# Autodesk Inventor assembly: AssemblyFullPrinter
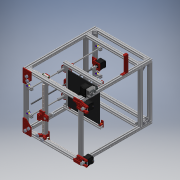
[picture p0: Inventor's stored thumbnail of the model, 180x180]
Saved by Autodesk Inventor 2018 (Build 220112000, 112)
## iProperties
Created: 2017-10-01
Part Number: AssemblyFullPrinter
Document SubType Name: Assembly
Designer: Jurjen
Author: Jurjen
## Documents named in this file (42)
- C:\Users\Jurjen\Documents\3D Printer\coreXY\AssemblyFullPrinter.iam
- C:\Users\Jurjen\Documents\3D Printer\coreXY\2020-350mm.ipt
- C:\Users\Jurjen\Documents\3D Printer\coreXY\2020-500mm.ipt
- C:\Users\Jurjen\Documents\3D Printer\coreXY\2020-corner-bracket.ipt
- C:\Users\Jurjen\Documents\3D Printer\coreXY\heated-bed.ipt
- C:\Users\Jurjen\Documents\3D Printer\coreXY\T8-lead-screw.ipt
- C:\Users\Jurjen\Documents\3D Printer\coreXY\motedis\GT2-Pulley-20-Teeth-5mm-Bore.ipt
- C:\Users\Jurjen\Documents\3D Printer\coreXY\motedis\Gt20.ipt
- C:\Users\Jurjen\Documents\3D Printer\coreXY\motedis\shaft-couple-flex.ipt
- C:\Users\Jurjen\Documents\3D Printer\coreXY\motedis\Motedis_SH8.ipt
- C:\Users\Jurjen\Documents\3D Printer\coreXY\rod-8mm.ipt
- C:\Users\Jurjen\Documents\3D Printer\coreXY\2020-260mm.ipt
- C:\Users\Jurjen\Documents\3D Printer\coreXY\2020-240mm.ipt
- C:\Users\Jurjen\Documents\3D Printer\coreXY\T8x2mm lead screw.ipt
- C:\Users\Jurjen\Documents\3D Printer\coreXY\OldhamCouplerBottom.ipt
- C:\Users\Jurjen\Documents\3D Printer\coreXY\OldhamCouplerMiddle.ipt
- C:\Users\Jurjen\Documents\3D Printer\coreXY\OldhamCouplerTop.ipt
- C:\Users\Jurjen\Documents\3D Printer\coreXY\M5-nut.ipt
- C:\Users\Jurjen\Documents\3D Printer\coreXY\nema17-mount-bottom-z-axis.ipt
- C:\Users\Jurjen\Documents\3D Printer\coreXY\bracket-GT2-left.ipt
- C:\Users\Jurjen\Documents\3D Printer\coreXY\M5x30mm.ipt
- C:\Users\Jurjen\Documents\3D Printer\coreXY\mount-heated-bed.ipt
- C:\Users\Jurjen\Documents\3D Printer\coreXY\bracket-GT2-right.ipt
- C:\Users\Jurjen\Documents\3D Printer\coreXY\spool-holder.ipt
- C:\Users\Jurjen\Documents\3D Printer\coreXY\17HM15-0904S\nema-17.ipt
- C:\Users\Jurjen\Documents\3D Printer\coreXY\nema17-mount-left.ipt
- C:\Users\Jurjen\Documents\3D Printer\coreXY\nema17-mount-right.ipt
- C:\Users\Jurjen\Documents\3D Printer\coreXY\LMF8LUU.ipt
- C:\Users\Jurjen\Documents\3D Printer\coreXY\holder-LMF8LUU-z-axis.ipt
- C:\Users\Jurjen\Documents\3D Printer\coreXY\MGN-12-rail.ipt
- C:\Users\Jurjen\Documents\3D Printer\coreXY\2020-320mm.ipt
- C:\Users\Jurjen\Documents\3D Printer\coreXY\x-carriage-2020.ipt
- C:\Users\Jurjen\Documents\3D Printer\coreXY\X-connectorLeft.ipt
- C:\Users\Jurjen\Documents\3D Printer\coreXY\X-connectorLeft_MIR.ipt
- C:\Users\Jurjen\Documents\3D Printer\coreXY\MGN-12-H-carriage.ipt
- C:\Users\Jurjen\Documents\3D Printer\coreXY\ED3V6.ipt
- C:\Users\Jurjen\Documents\3D Printer\coreXY\x-carriage.ipt
- C:\Users\Jurjen\Documents\3D Printer\coreXY\x-carriage-holder.ipt
- C:\Users\Jurjen\Documents\3D Printer\coreXY\holder-GT2-x-carriage-left.ipt
- C:\Users\Jurjen\Documents\3D Printer\coreXY\M5x35mm-crosshead.ipt
- C:\Users\Jurjen\Documents\3D Printer\coreXY\extruder\e3d titan.iam
- C:\Users\Jurjen\Documents\3D Printer\coreXY\mount-extruder.ipt
## Components (122 placed, 41 different names)
1. spool-holder:1 — Mate:287, Mate:288, Flush:54
2. 2020-500mm:1 — Mate:1, Flush:2, Flush:14, Flush:17, Mate:11, Mate:85, Flush:37, Mate:90, Mate:92, Mate:93, Mate:94, Mate:131, Mate:132, Mate:163, Mate:165, Mate:166, Mate:168, Mate:287, Mate:288, Flush:54, Mate:348, Mate:359, Mate:360, Mate:434, Flush:78, Mate:459, Mate:471, Mate:472, Mate:473
3. 2020-500mm:2 — Mate:2, Flush:1, Flush:13, Flush:14, Mate:12, Flush:23, Mate:75, Mate:77, Mate:79, Mate:80, Mate:133, Mate:135, Mate:151, Mate:152, Mate:154, Mate:156, Mate:346, Flush:63, Mate:362, Mate:439, Mate:455
4. 2020-500mm:3 — Mate:8, Flush:12, Flush:13, Flush:15, Mate:9, Flush:30, Mate:82, Mate:83, Mate:86, Flush:39, Mate:136, Mate:138, Mate:140, Mate:141, Mate:149, Mate:150, Mate:342, Flush:62, Flush:67, Mate:367, Flush:82, Mate:456
5. 2020-500mm:4 — Mate:7, Flush:15, Mate:10, Flush:27, Mate:142, Mate:144, Mate:145, Mate:147, Mate:157, Mate:158, Mate:160, Mate:162, Flush:64, Mate:354, Flush:65, Mate:447, Mate:450
6. 2020-320mm:3 — Mate:353, Mate:354, Mate:355, Mate:356, Flush:65, Flush:66, Mate:357, Mate:358, Mate:368, Mate:369, Mate:373, Mate:374, Mate:388, Flush:73, Mate:446, Mate:448, Mate:460, Mate:461
7. 2020-320mm:4 — Flush:67, Mate:362, Mate:363, Mate:364, Flush:68, Mate:366, Flush:69, Mate:371, Mate:372, Mate:385, Mate:386, Mate:387, Flush:72, Mate:453, Mate:454, Mate:457, Mate:458
8. 2020-350mm:1 — Mate:1, Mate:2, Flush:1, Flush:2, Mate:19, Mate:23, Mate:76, Mate:95, Mate:294, Mate:303, Mate:304, Mate:307, Mate:308, Flush:66, Flush:68
9. 2020-350mm:4 — Mate:7, Mate:8, Flush:12, Mate:16, Mate:26, Flush:27, Mate:60, Mate:61, Mate:64, Mate:65, Mate:66, Mate:67, Mate:239, Mate:277, Mate:279, Flush:53, Mate:337, Flush:70, Mate:449, Mate:452
10. 2020-corner-bracket:1 — Mate:16, Mate:356, Mate:452
11. 2020-corner-bracket:2 — Mate:23, Mate:363, Mate:364
12. 2020-corner-bracket:3 — Mate:19, Mate:357, Mate:358
13. 2020-corner-bracket:4 — Mate:26, Mate:385, Mate:386
14. 2020-corner-bracket:10 — Mate:75, Mate:76, Mate:77
15. 2020-corner-bracket:13 — Mate:93, Mate:94, Mate:95, Mate:359
16. 2020-corner-bracket:33 — Mate:449, Mate:450
17. 2020-corner-bracket:34 — Mate:446, Mate:447, Mate:448
18. 2020-corner-bracket:35 — Mate:453, Mate:454, Mate:455
19. 2020-corner-bracket:36 — Mate:456, Mate:457, Mate:458
20. 2020-corner-bracket:37 — Mate:459, Mate:460, Mate:461
21. 2020-320mm:1 — Mate:347, Flush:64, Mate:348, Mate:349, Mate:350, Mate:351, Mate:352
22. 2020-320mm:2 — Mate:338, Mate:339, Mate:341, Flush:61, Mate:342, Mate:343, Mate:344, Flush:62, Mate:345, Mate:346, Flush:63, Mate:445
23. 2020-350mm:5 — Flush:17, Mate:11, Mate:12, Mate:31, Mate:35, Flush:23, Mate:78, Mate:89, Mate:91, Mate:340, Flush:61
24. 2020-350mm:6 — Mate:9, Mate:10, Mate:27, Mate:28, Mate:29, Mate:30, Mate:34, Mate:38, Flush:30, Mate:62, Mate:63, Mate:68, Mate:69, Mate:70, Mate:71, Mate:72, Mate:139, Mate:146, Mate:230, Flush:59, Flush:60
25. 2020-corner-bracket:5 — Mate:27, Mate:38, Mate:351
26. 2020-corner-bracket:6 — Mate:28, Mate:34, Mate:343, Mate:345
27. 2020-corner-bracket:7 — Mate:30, Mate:35, Mate:338, Mate:339, Mate:340
28. 2020-corner-bracket:8 — Mate:29, Mate:31, Mate:349
29. 2020-corner-bracket:9 — Mate:78, Mate:79, Mate:80
30. 2020-corner-bracket:11 — Mate:82, Mate:83, Mate:344
31. 2020-corner-bracket:12 — Mate:89, Mate:90, Mate:91, Mate:92
32. 2020-corner-bracket:16 — Mate:139, Mate:140, Mate:141
33. 2020-corner-bracket:21 — Mate:145, Mate:146, Mate:147
34. 2020-corner-bracket:23 — Mate:151, Mate:152, Mate:341
35. 2020-corner-bracket:25 — Mate:157, Mate:158, Mate:347, Mate:352
36. 2020-corner-bracket:28 — Mate:166, Mate:168, Mate:350
37. 2020-350mm:10 — Mate:85, Flush:37, Mate:130, Mate:134, Mate:169, Mate:171, Mate:178, Mate:181, Flush:79
38. 2020-350mm:11 — Mate:86, Flush:39, Mate:137, Mate:143, Mate:174, Mate:176, Mate:179, Flush:80, Flush:81
39. 2020-320mm:5 — Mate:434, Mate:435, Flush:78, Mate:436, Flush:79, Flush:80, Mate:437, Mate:438, Mate:444
40. 2020-320mm:6 — Flush:81, Mate:439, Mate:440, Mate:441, Flush:82, Mate:442, Mate:443, Mate:445
41. 2020-corner-bracket:17 — Mate:133, Mate:134, Mate:135
42. 2020-corner-bracket:18 — Mate:130, Mate:131, Mate:132
43. 2020-corner-bracket:19 — Mate:136, Mate:137, Mate:138
44. 2020-corner-bracket:20 — Mate:142, Mate:143, Mate:144
45. 2020-corner-bracket:22 — Mate:149, Mate:150, Mate:442
46. 2020-corner-bracket:24 — Mate:154, Mate:156, Mate:440
47. 2020-corner-bracket:26 — Mate:160, Mate:162, Mate:437
48. 2020-corner-bracket:27 — Mate:163, Mate:165, Mate:436
49. 2020-corner-bracket:29 — Mate:169, Mate:178, Mate:441
50. 2020-corner-bracket:30 — Mate:171, Mate:181, Mate:435
51. 2020-corner-bracket:31 — Mate:174, Mate:438, Mate:444
52. 2020-corner-bracket:32 — Mate:176, Mate:179, Mate:443
53. 2020-corner-bracket:14 — Mate:122, Mate:123, Mate:124
54. 2020-corner-bracket:15 — Mate:119, Mate:120, Mate:121, Flush:49
55. shaft-couple-flex:1 — Mate:59, Mate:114, Mate:293
56. LMF8LUU:1 — Mate:313, Mate:317, Mate:318, Mate:320
57. LMF8LUU:2 — Mate:314, Mate:324, Mate:326, Mate:327
58. holder-LMF8LUU-z-axis:1 — Mate:316, Mate:317, Mate:318, Mate:319, Mate:320, Mate:321, Mate:322
59. holder-LMF8LUU-z-axis:2 — Mate:324, Mate:326, Mate:327, Mate:328, Mate:329, Mate:332
60. T8-lead-screw:1 — Mate:59, Mate:114, Mate:115, Mate:116, Mate:117, Mate:118, Mate:315
61. nema-17:1 — Mate:290, Mate:291, Mate:292, Mate:293, Mate:315
62. nema17-mount-bottom-z-axis:1 — Mate:230, Mate:290, Mate:291, Mate:292, Flush:59, Flush:60, Mate:330, Mate:331
63. rod-8mm:1 — Mate:73, Flush:34, Mate:314
64. rod-8mm:2 — Mate:74, Flush:35, Mate:313, Mate:316
65. heated-bed:1 — Mate:267, Mate:269, Mate:272, Mate:275, Mate:276
66. 2020-260mm:1 — Mate:109, Flush:45, Flush:46, Mate:123, Mate:265, Mate:266, Flush:52, Mate:270, Mate:271
67. 2020-260mm:2 — Mate:107, Flush:45, Flush:47, Mate:119, Flush:49, Mate:263, Mate:264, Flush:51, Mate:273, Mate:274
68. 2020-240mm:1 — Mate:103, Mate:104, Mate:105, Mate:107, Mate:109, Flush:46, Flush:47, Mate:110, Mate:120, Mate:121, Mate:122, Mate:124, Mate:319, Mate:321, Mate:322, Mate:328, Mate:329, Mate:332
69. mount-heated-bed:1 — Mate:263, Mate:264, Flush:51, Mate:267, Mate:276
70. mount-heated-bed:2 — Mate:265, Mate:266, Flush:52, Mate:269
71. mount-heated-bed:3 — Mate:270, Mate:271, Mate:272
72. mount-heated-bed:4 — Mate:273, Mate:274, Mate:275
73. Gt20:7 — Mate:424, Mate:433, Flush:76
74. Gt20:8 — Mate:423, Mate:427, Flush:77
75. MGN-12-rail:2 — Mate:373, Mate:374, Mate:388, Mate:394, Mate:395, Flush:73
76. MGN-12-rail:3 — Mate:371, Mate:372, Mate:387, Mate:392, Mate:393, Flush:72
77. MGN-12-H-carriage:1 — Mate:392, Mate:393, Mate:399, Mate:415
78. MGN-12-H-carriage:3 — Mate:394, Mate:395, Mate:396, Mate:397, Mate:398
79. GT2-Pulley-20-Teeth-5mm-Bore:2 — Mate:312, Flush:75
80. GT2-Pulley-20-Teeth-5mm-Bore:1 — Mate:297, Flush:56
81. bracket-GT2-right:1 — Mate:277, Mate:279, Mate:280, Mate:281, Mate:283, Mate:284, Mate:285, Mate:286, Flush:53, Mate:353, Mate:355
82. Gt20:5 — Mate:240, Mate:241, Flush:56, Mate:419, Flush:77
83. Gt20:6 — Mate:242, Mate:243, Mate:262, Flush:76
84. M5-nut:6 — Mate:260, Mate:283
85. bracket-GT2-left:1 — Mate:237, Mate:238, Mate:239, Mate:245, Mate:247, Mate:262, Mate:366, Mate:367, Flush:70, Mate:419
86. M5-nut:3 — Mate:244, Mate:245
87. M5-nut:5 — Mate:246, Mate:247
88. M5x30mm:1 — Mate:237, Mate:240, Mate:241, Mate:244
89. M5x30mm:2 — Mate:238, Mate:242, Mate:243, Mate:246
90. M5x30mm:3 — Mate:254, Mate:256, Mate:260, Mate:281
91. M5x30mm:4 — Mate:255, Mate:257, Mate:258, Mate:280
92. Gt20:2 — Mate:254, Mate:256, Mate:286, Flush:75
93. Gt20:4 — Mate:255, Mate:257, Mate:285
94. M5-nut:2 — Mate:258, Mate:284
95. nema-17:2 — Mate:297, Mate:298, Mate:299, Mate:300, Flush:57
96. nema-17:3 — Mate:309, Mate:310, Flush:58, Mate:311, Mate:312
97. nema17-mount-left:1 — Mate:294, Mate:298, Mate:299, Mate:300, Flush:57, Mate:303, Mate:304, Flush:69
98. nema17-mount-right:1 — Mate:307, Mate:308, Mate:309, Mate:310, Flush:58, Mate:311, Mate:360, Mate:368, Mate:369
99. e3d titan:1 [sub-assembly] — Mate:465, Mate:466, Mate:470
100. mount-extruder:1 — Mate:465, Mate:466, Mate:467, Mate:468, Mate:469, Mate:470, Mate:471, Mate:472, Mate:473
101. nema-17:4 — Mate:467, Mate:468, Mate:469
102. Motedis_SH8:1 — Mate:63, Mate:71, Mate:72, Flush:33, Mate:331
103. Motedis_SH8:2 — Mate:62, Mate:68, Mate:69, Mate:70, Flush:32, Mate:330
104. Motedis_SH8:3 — Mate:61, Mate:64, Mate:65, Flush:33, Mate:74, Flush:35
105. Motedis_SH8:4 — Mate:60, Mate:66, Mate:67, Flush:32, Mate:73, Flush:34
106. T8x2mm lead screw:1 — Mate:100, Mate:118
107. OldhamCouplerBottom:1 — Mate:99, Flush:43, Mate:100, Mate:117
108. OldhamCouplerMiddle:1 — Mate:99, Flush:43, Flush:44, Mate:102, Mate:115
109. OldhamCouplerTop:1 — Flush:44, Mate:102, Mate:103, Mate:104, Mate:105, Mate:110, Mate:116, Mate:337
110. MGN-12-rail:1 — Mate:381, Mate:389, Mate:390, Mate:391, Flush:71
111. x-carriage-2020:1 — Mate:377, Mate:381, Mate:384, Mate:389, Flush:71, Mate:409, Mate:410, Mate:411, Mate:421, Mate:422, Mate:432
112. X-connectorLeft:1 — Mate:377, Mate:396, Mate:397, Mate:398, Mate:410, Mate:411
113. X-connectorLeft_MIR:1 — Mate:384, Mate:399, Mate:409, Mate:415
114. MGN-12-H-carriage:2 — Mate:390, Mate:391, Mate:402, Mate:403, Mate:404
115. x-carriage-holder:1 — Mate:406, Mate:407, Mate:408
116. x-carriage:1 — Mate:402, Mate:403, Mate:404, Mate:405, Mate:406, Mate:407, Mate:408, Flush:74
117. holder-GT2-x-carriage-left:1 — Mate:421, Mate:422, Mate:425, Mate:426, Mate:429, Mate:431, Mate:432
118. M5-nut:7 — Mate:428, Mate:429
119. M5x35mm-crosshead:1 — Mate:423, Mate:426, Mate:427, Mate:428
120. M5-nut:8 — Mate:430, Mate:431
121. M5x35mm-crosshead:2 — Mate:424, Mate:425, Mate:430, Mate:433
122. ED3V6:1 — Mate:405, Flush:74
## Relationships (356: Mate 303, Flush 53)
- Mate:1: 2020-500mm:1 ↔ 2020-350mm:1
- Mate:2: 2020-500mm:2 ↔ 2020-350mm:1
- Flush:1: 2020-500mm:2 ↔ 2020-350mm:1
- Flush:2: 2020-500mm:1 ↔ 2020-350mm:1
- Mate:7: 2020-500mm:4 ↔ 2020-350mm:4
- Mate:8: 2020-500mm:3 ↔ 2020-350mm:4
- Flush:12: 2020-500mm:3 ↔ 2020-350mm:4
- Flush:13: 2020-500mm:2 ↔ 2020-500mm:3
- Flush:14: 2020-500mm:1 ↔ 2020-500mm:2
- Flush:15: 2020-500mm:3 ↔ 2020-500mm:4
- Mate:9: 2020-500mm:3 ↔ 2020-350mm:6
- Mate:10: 2020-500mm:4 ↔ 2020-350mm:6
- Flush:17: 2020-500mm:1 ↔ 2020-350mm:5
- Mate:11: 2020-500mm:1 ↔ 2020-350mm:5
- Mate:12: 2020-500mm:2 ↔ 2020-350mm:5
- Mate:16: 2020-350mm:4 ↔ 2020-corner-bracket:1
- Mate:19: 2020-350mm:1 ↔ 2020-corner-bracket:3
- Mate:23: 2020-350mm:1 ↔ 2020-corner-bracket:2
- Mate:26: 2020-350mm:4 ↔ 2020-corner-bracket:4
- Mate:27: 2020-350mm:6 ↔ 2020-corner-bracket:5
- Mate:28: 2020-350mm:6 ↔ 2020-corner-bracket:6
- Mate:29: 2020-350mm:6 ↔ 2020-corner-bracket:8
- Mate:30: 2020-350mm:6 ↔ 2020-corner-bracket:7
- Mate:31: 2020-350mm:5 ↔ 2020-corner-bracket:8
- Mate:34: 2020-350mm:6 ↔ 2020-corner-bracket:6
- Mate:35: 2020-350mm:5 ↔ 2020-corner-bracket:7
- Mate:38: 2020-350mm:6 ↔ 2020-corner-bracket:5
- Flush:23: 2020-500mm:2 ↔ 2020-350mm:5
- Flush:27: 2020-500mm:4 ↔ 2020-350mm:4
- Flush:30: 2020-500mm:3 ↔ 2020-350mm:6
- Mate:59 (-8 mm): shaft-couple-flex:1 ↔ T8-lead-screw:1
- Mate:60: 2020-350mm:4 ↔ Motedis_SH8:4
- Mate:61: 2020-350mm:4 ↔ Motedis_SH8:3
- Mate:62: 2020-350mm:6 ↔ Motedis_SH8:2
- Mate:63: 2020-350mm:6 ↔ Motedis_SH8:1
- Mate:64: 2020-350mm:4 ↔ Motedis_SH8:3
- Mate:65: 2020-350mm:4 ↔ Motedis_SH8:3
- Mate:66: 2020-350mm:4 ↔ Motedis_SH8:4
- Mate:67: 2020-350mm:4 ↔ Motedis_SH8:4
- Mate:68: 2020-350mm:6 ↔ Motedis_SH8:2
- Mate:69: 2020-350mm:6 ↔ Motedis_SH8:2
- Mate:70: 2020-350mm:6 ↔ Motedis_SH8:2
- Flush:32: Motedis_SH8:2 ↔ Motedis_SH8:4
- Mate:71: 2020-350mm:6 ↔ Motedis_SH8:1
- Mate:72: 2020-350mm:6 ↔ Motedis_SH8:1
- Flush:33: Motedis_SH8:1 ↔ Motedis_SH8:3
- Mate:73: rod-8mm:1 ↔ Motedis_SH8:4
- Mate:74: rod-8mm:2 ↔ Motedis_SH8:3
- Flush:34 (-5 mm): rod-8mm:1 ↔ Motedis_SH8:4
- Flush:35 (-5 mm): rod-8mm:2 ↔ Motedis_SH8:3
- Mate:75: 2020-500mm:2 ↔ 2020-corner-bracket:10
- Mate:76: 2020-350mm:1 ↔ 2020-corner-bracket:10
- Mate:77: 2020-500mm:2 ↔ 2020-corner-bracket:10
- Mate:78: 2020-350mm:5 ↔ 2020-corner-bracket:9
- Mate:79: 2020-500mm:2 ↔ 2020-corner-bracket:9
- Mate:80: 2020-500mm:2 ↔ 2020-corner-bracket:9
- Mate:82: 2020-500mm:3 ↔ 2020-corner-bracket:11
- Mate:83: 2020-500mm:3 ↔ 2020-corner-bracket:11
- Mate:85: 2020-500mm:1 ↔ 2020-350mm:10
- Flush:37: 2020-500mm:1 ↔ 2020-350mm:10
- Mate:86: 2020-500mm:3 ↔ 2020-350mm:11
- Flush:39: 2020-500mm:3 ↔ 2020-350mm:11
- Mate:89: 2020-350mm:5 ↔ 2020-corner-bracket:12
- Mate:90: 2020-500mm:1 ↔ 2020-corner-bracket:12
- Mate:91: 2020-350mm:5 ↔ 2020-corner-bracket:12
- Mate:92: 2020-500mm:1 ↔ 2020-corner-bracket:12
- Mate:93: 2020-500mm:1 ↔ 2020-corner-bracket:13
- Mate:94: 2020-500mm:1 ↔ 2020-corner-bracket:13
- Mate:95: 2020-350mm:1 ↔ 2020-corner-bracket:13
- Mate:99: OldhamCouplerBottom:1 ↔ OldhamCouplerMiddle:1
- Flush:43: OldhamCouplerBottom:1 ↔ OldhamCouplerMiddle:1
- Mate:100: T8x2mm lead screw:1 ↔ OldhamCouplerBottom:1
- Flush:44: OldhamCouplerMiddle:1 ↔ OldhamCouplerTop:1
- Mate:102: OldhamCouplerMiddle:1 ↔ OldhamCouplerTop:1
- Mate:103: 2020-240mm:1 ↔ OldhamCouplerTop:1
- Mate:104: 2020-240mm:1 ↔ OldhamCouplerTop:1
- Mate:105: 2020-240mm:1 ↔ OldhamCouplerTop:1
- Mate:107: 2020-260mm:2 ↔ 2020-240mm:1
- Mate:109: 2020-260mm:1 ↔ 2020-240mm:1
- Flush:45: 2020-260mm:1 ↔ 2020-260mm:2
- Flush:46: 2020-260mm:1 ↔ 2020-240mm:1
- Flush:47: 2020-260mm:2 ↔ 2020-240mm:1
- Mate:110: 2020-240mm:1 ↔ OldhamCouplerTop:1
- Mate:114: shaft-couple-flex:1 ↔ T8-lead-screw:1
- Mate:115: T8-lead-screw:1 ↔ OldhamCouplerMiddle:1
- Mate:116: T8-lead-screw:1 ↔ OldhamCouplerTop:1
- Mate:117: T8-lead-screw:1 ↔ OldhamCouplerBottom:1
- Mate:118: T8-lead-screw:1 ↔ T8x2mm lead screw:1
- Mate:119: 2020-corner-bracket:15 ↔ 2020-260mm:2
- Mate:120: 2020-corner-bracket:15 ↔ 2020-240mm:1
- Mate:121: 2020-corner-bracket:15 ↔ 2020-240mm:1
- Flush:49: 2020-corner-bracket:15 ↔ 2020-260mm:2
- Mate:122: 2020-corner-bracket:14 ↔ 2020-240mm:1
- Mate:123: 2020-corner-bracket:14 ↔ 2020-260mm:1
- Mate:124: 2020-corner-bracket:14 ↔ 2020-240mm:1
- Mate:130: 2020-350mm:10 ↔ 2020-corner-bracket:18
- Mate:131: 2020-500mm:1 ↔ 2020-corner-bracket:18
- Mate:132: 2020-500mm:1 ↔ 2020-corner-bracket:18
- Mate:133: 2020-500mm:2 ↔ 2020-corner-bracket:17
- Mate:134: 2020-350mm:10 ↔ 2020-corner-bracket:17
- Mate:135: 2020-500mm:2 ↔ 2020-corner-bracket:17
- Mate:136: 2020-500mm:3 ↔ 2020-corner-bracket:19
- Mate:137: 2020-350mm:11 ↔ 2020-corner-bracket:19
- Mate:138: 2020-500mm:3 ↔ 2020-corner-bracket:19
- Mate:139: 2020-350mm:6 ↔ 2020-corner-bracket:16
- Mate:140: 2020-500mm:3 ↔ 2020-corner-bracket:16
- Mate:141: 2020-500mm:3 ↔ 2020-corner-bracket:16
- Mate:142: 2020-500mm:4 ↔ 2020-corner-bracket:20
- Mate:143: 2020-350mm:11 ↔ 2020-corner-bracket:20
- Mate:144: 2020-500mm:4 ↔ 2020-corner-bracket:20
- Mate:145: 2020-500mm:4 ↔ 2020-corner-bracket:21
- Mate:146: 2020-350mm:6 ↔ 2020-corner-bracket:21
- Mate:147: 2020-500mm:4 ↔ 2020-corner-bracket:21
- Mate:149: 2020-500mm:3 ↔ 2020-corner-bracket:22
- Mate:150: 2020-500mm:3 ↔ 2020-corner-bracket:22
- Mate:151: 2020-500mm:2 ↔ 2020-corner-bracket:23
- Mate:152: 2020-500mm:2 ↔ 2020-corner-bracket:23
- Mate:154: 2020-500mm:2 ↔ 2020-corner-bracket:24
- Mate:156: 2020-500mm:2 ↔ 2020-corner-bracket:24
- Mate:157: 2020-500mm:4 ↔ 2020-corner-bracket:25
- Mate:158: 2020-500mm:4 ↔ 2020-corner-bracket:25
- Mate:160: 2020-500mm:4 ↔ 2020-corner-bracket:26
- Mate:162: 2020-500mm:4 ↔ 2020-corner-bracket:26
- Mate:163: 2020-500mm:1 ↔ 2020-corner-bracket:27
- Mate:165: 2020-500mm:1 ↔ 2020-corner-bracket:27
- Mate:166: 2020-500mm:1 ↔ 2020-corner-bracket:28
- Mate:168: 2020-500mm:1 ↔ 2020-corner-bracket:28
- Mate:169: 2020-350mm:10 ↔ 2020-corner-bracket:29
- Mate:171: 2020-350mm:10 ↔ 2020-corner-bracket:30
- Mate:174: 2020-350mm:11 ↔ 2020-corner-bracket:31
- Mate:176: 2020-350mm:11 ↔ 2020-corner-bracket:32
- Mate:178: 2020-350mm:10 ↔ 2020-corner-bracket:29
- Mate:179: 2020-350mm:11 ↔ 2020-corner-bracket:32
- Mate:181: 2020-350mm:10 ↔ 2020-corner-bracket:30
- Mate:230: 2020-350mm:6 ↔ nema17-mount-bottom-z-axis:1
- Mate:237: bracket-GT2-left:1 ↔ M5x30mm:1
- Mate:238: bracket-GT2-left:1 ↔ M5x30mm:2
- Mate:239: 2020-350mm:4 ↔ bracket-GT2-left:1
- Mate:240: Gt20:5 ↔ M5x30mm:1
- Mate:241: Gt20:5 ↔ M5x30mm:1
- Mate:242: Gt20:6 ↔ M5x30mm:2
- Mate:243: Gt20:6 ↔ M5x30mm:2
- Mate:244: M5-nut:3 ↔ M5x30mm:1
- Mate:245: bracket-GT2-left:1 ↔ M5-nut:3
- Mate:246: M5-nut:5 ↔ M5x30mm:2
- Mate:247: bracket-GT2-left:1 ↔ M5-nut:5
- Mate:254: M5x30mm:3 ↔ Gt20:2
- Mate:255: M5x30mm:4 ↔ Gt20:4
- Mate:256: M5x30mm:3 ↔ Gt20:2
- Mate:257: M5x30mm:4 ↔ Gt20:4
- Mate:258: M5x30mm:4 ↔ M5-nut:2
- Mate:260: M5-nut:6 ↔ M5x30mm:3
- Mate:262: Gt20:6 ↔ bracket-GT2-left:1
- Mate:263: 2020-260mm:2 ↔ mount-heated-bed:1
- Mate:264: 2020-260mm:2 ↔ mount-heated-bed:1
- Flush:51: 2020-260mm:2 ↔ mount-heated-bed:1
- Mate:265: 2020-260mm:1 ↔ mount-heated-bed:2
- Mate:266: 2020-260mm:1 ↔ mount-heated-bed:2
- Flush:52: 2020-260mm:1 ↔ mount-heated-bed:2
- Mate:267: heated-bed:1 ↔ mount-heated-bed:1
- Mate:269: heated-bed:1 ↔ mount-heated-bed:2
- Mate:270: 2020-260mm:1 ↔ mount-heated-bed:3
- Mate:271: 2020-260mm:1 ↔ mount-heated-bed:3
- Mate:272: heated-bed:1 ↔ mount-heated-bed:3
- Mate:273: 2020-260mm:2 ↔ mount-heated-bed:4
- Mate:274: 2020-260mm:2 ↔ mount-heated-bed:4
- Mate:275: heated-bed:1 ↔ mount-heated-bed:4
- Mate:276 (20 mm): heated-bed:1 ↔ mount-heated-bed:1
- Mate:277: 2020-350mm:4 ↔ bracket-GT2-right:1
- Mate:279: 2020-350mm:4 ↔ bracket-GT2-right:1
- Mate:280: bracket-GT2-right:1 ↔ M5x30mm:4
- Mate:281: bracket-GT2-right:1 ↔ M5x30mm:3
- Mate:283: bracket-GT2-right:1 ↔ M5-nut:6
- Mate:284: bracket-GT2-right:1 ↔ M5-nut:2
- Mate:285: bracket-GT2-right:1 ↔ Gt20:4
- Mate:286: bracket-GT2-right:1 ↔ Gt20:2
- Flush:53: 2020-350mm:4 ↔ bracket-GT2-right:1
- Mate:287: spool-holder:1 ↔ 2020-500mm:1
- Mate:288: spool-holder:1 ↔ 2020-500mm:1
- Flush:54: spool-holder:1 ↔ 2020-500mm:1
- Mate:290: nema-17:1 ↔ nema17-mount-bottom-z-axis:1
- Mate:291: nema-17:1 ↔ nema17-mount-bottom-z-axis:1
- Mate:292: nema-17:1 ↔ nema17-mount-bottom-z-axis:1
- Mate:293 (-8 mm): shaft-couple-flex:1 ↔ nema-17:1
- Mate:294: 2020-350mm:1 ↔ nema17-mount-left:1
- Mate:297: GT2-Pulley-20-Teeth-5mm-Bore:1 ↔ nema-17:2
- Flush:56: GT2-Pulley-20-Teeth-5mm-Bore:1 ↔ Gt20:5
- Mate:298: nema-17:2 ↔ nema17-mount-left:1
- Mate:299: nema-17:2 ↔ nema17-mount-left:1
- Mate:300: nema-17:2 ↔ nema17-mount-left:1
- Flush:57: nema-17:2 ↔ nema17-mount-left:1
- Mate:303: 2020-350mm:1 ↔ nema17-mount-left:1
- Mate:304: 2020-350mm:1 ↔ nema17-mount-left:1
- Mate:307: 2020-350mm:1 ↔ nema17-mount-right:1
- Mate:308: 2020-350mm:1 ↔ nema17-mount-right:1
- Mate:309: nema-17:3 ↔ nema17-mount-right:1
- Mate:310: nema-17:3 ↔ nema17-mount-right:1
- Flush:58: nema-17:3 ↔ nema17-mount-right:1
- Mate:311: nema-17:3 ↔ nema17-mount-right:1
- Mate:312: GT2-Pulley-20-Teeth-5mm-Bore:2 ↔ nema-17:3
- Mate:313: LMF8LUU:1 ↔ rod-8mm:2
- Mate:314: LMF8LUU:2 ↔ rod-8mm:1
- Flush:59: 2020-350mm:6 ↔ nema17-mount-bottom-z-axis:1
- Flush:60: 2020-350mm:6 ↔ nema17-mount-bottom-z-axis:1
- Mate:315: T8-lead-screw:1 ↔ nema-17:1
- Mate:316: holder-LMF8LUU-z-axis:1 ↔ rod-8mm:2
- Mate:317: LMF8LUU:1 ↔ holder-LMF8LUU-z-axis:1
- Mate:318: LMF8LUU:1 ↔ holder-LMF8LUU-z-axis:1
- Mate:319: holder-LMF8LUU-z-axis:1 ↔ 2020-240mm:1
- Mate:320: LMF8LUU:1 ↔ holder-LMF8LUU-z-axis:1
- Mate:321: holder-LMF8LUU-z-axis:1 ↔ 2020-240mm:1
- Mate:322: holder-LMF8LUU-z-axis:1 ↔ 2020-240mm:1
- Mate:324: LMF8LUU:2 ↔ holder-LMF8LUU-z-axis:2
- Mate:326: LMF8LUU:2 ↔ holder-LMF8LUU-z-axis:2
- Mate:327: LMF8LUU:2 ↔ holder-LMF8LUU-z-axis:2
- Mate:328: holder-LMF8LUU-z-axis:2 ↔ 2020-240mm:1
- Mate:329: holder-LMF8LUU-z-axis:2 ↔ 2020-240mm:1
- Mate:330 (40 mm): nema17-mount-bottom-z-axis:1 ↔ Motedis_SH8:2
- Mate:331 (40 mm): nema17-mount-bottom-z-axis:1 ↔ Motedis_SH8:1
- Mate:332: holder-LMF8LUU-z-axis:2 ↔ 2020-240mm:1
- Mate:337: 2020-350mm:4 ↔ OldhamCouplerTop:1
- Mate:338: 2020-320mm:2 ↔ 2020-corner-bracket:7
- Mate:339: 2020-320mm:2 ↔ 2020-corner-bracket:7
- Mate:340: 2020-350mm:5 ↔ 2020-corner-bracket:7
- Mate:341: 2020-320mm:2 ↔ 2020-corner-bracket:23
- Flush:61: 2020-320mm:2 ↔ 2020-350mm:5
- Mate:342: 2020-500mm:3 ↔ 2020-320mm:2
- Mate:343: 2020-320mm:2 ↔ 2020-corner-bracket:6
- Mate:344: 2020-320mm:2 ↔ 2020-corner-bracket:11
- Flush:62: 2020-500mm:3 ↔ 2020-320mm:2
- Mate:345: 2020-320mm:2 ↔ 2020-corner-bracket:6
- Mate:346: 2020-500mm:2 ↔ 2020-320mm:2
- Flush:63: 2020-500mm:2 ↔ 2020-320mm:2
- Mate:347: 2020-320mm:1 ↔ 2020-corner-bracket:25
- Flush:64: 2020-500mm:4 ↔ 2020-320mm:1
- Mate:348: 2020-500mm:1 ↔ 2020-320mm:1
- Mate:349: 2020-320mm:1 ↔ 2020-corner-bracket:8
- Mate:350: 2020-320mm:1 ↔ 2020-corner-bracket:28
- Mate:351: 2020-320mm:1 ↔ 2020-corner-bracket:5
- Mate:352: 2020-320mm:1 ↔ 2020-corner-bracket:25
- Mate:353: 2020-320mm:3 ↔ bracket-GT2-right:1
- Mate:354: 2020-500mm:4 ↔ 2020-320mm:3
- Mate:355: 2020-320mm:3 ↔ bracket-GT2-right:1
- Mate:356: 2020-320mm:3 ↔ 2020-corner-bracket:1
- Flush:65: 2020-500mm:4 ↔ 2020-320mm:3
- Flush:66: 2020-320mm:3 ↔ 2020-350mm:1
- Mate:357: 2020-320mm:3 ↔ 2020-corner-bracket:3
- Mate:358: 2020-320mm:3 ↔ 2020-corner-bracket:3
- Mate:359: 2020-500mm:1 ↔ 2020-corner-bracket:13
- Mate:360: 2020-500mm:1 ↔ nema17-mount-right:1
- Flush:67: 2020-500mm:3 ↔ 2020-320mm:4
- Mate:362: 2020-500mm:2 ↔ 2020-320mm:4
- Mate:363: 2020-320mm:4 ↔ 2020-corner-bracket:2
- Mate:364: 2020-320mm:4 ↔ 2020-corner-bracket:2
- Flush:68: 2020-320mm:4 ↔ 2020-350mm:1
- Mate:366: 2020-320mm:4 ↔ bracket-GT2-left:1
- Mate:367: 2020-500mm:3 ↔ bracket-GT2-left:1
- Mate:368: 2020-320mm:3 ↔ nema17-mount-right:1
- Mate:369: 2020-320mm:3 ↔ nema17-mount-right:1
- Flush:69: 2020-320mm:4 ↔ nema17-mount-left:1
- Mate:371: 2020-320mm:4 ↔ MGN-12-rail:3
- Mate:372: 2020-320mm:4 ↔ MGN-12-rail:3
- Mate:373: 2020-320mm:3 ↔ MGN-12-rail:2
- Mate:374: 2020-320mm:3 ↔ MGN-12-rail:2
- Flush:70: 2020-350mm:4 ↔ bracket-GT2-left:1
- Mate:377: x-carriage-2020:1 ↔ X-connectorLeft:1
- Mate:381: MGN-12-rail:1 ↔ x-carriage-2020:1
- Mate:384: x-carriage-2020:1 ↔ X-connectorLeft_MIR:1
- Mate:385: 2020-320mm:4 ↔ 2020-corner-bracket:4
- Mate:386: 2020-320mm:4 ↔ 2020-corner-bracket:4
- Mate:387: 2020-320mm:4 ↔ MGN-12-rail:3
- Mate:388: 2020-320mm:3 ↔ MGN-12-rail:2
- Mate:389: MGN-12-rail:1 ↔ x-carriage-2020:1
- Mate:390: MGN-12-rail:1 ↔ MGN-12-H-carriage:2
- Mate:391: MGN-12-rail:1 ↔ MGN-12-H-carriage:2
- Mate:392: MGN-12-rail:3 ↔ MGN-12-H-carriage:1
- Mate:393: MGN-12-rail:3 ↔ MGN-12-H-carriage:1
- Mate:394: MGN-12-rail:2 ↔ MGN-12-H-carriage:3
- Mate:395: MGN-12-rail:2 ↔ MGN-12-H-carriage:3
- Mate:396: MGN-12-H-carriage:3 ↔ X-connectorLeft:1
- Mate:397: MGN-12-H-carriage:3 ↔ X-connectorLeft:1
- Mate:398: MGN-12-H-carriage:3 ↔ X-connectorLeft:1
- Mate:399: MGN-12-H-carriage:1 ↔ X-connectorLeft_MIR:1
- Flush:71: MGN-12-rail:1 ↔ x-carriage-2020:1
- Flush:72: 2020-320mm:4 ↔ MGN-12-rail:3
- Flush:73: 2020-320mm:3 ↔ MGN-12-rail:2
- Mate:402: MGN-12-H-carriage:2 ↔ x-carriage:1
- Mate:403: MGN-12-H-carriage:2 ↔ x-carriage:1
- Mate:404: MGN-12-H-carriage:2 ↔ x-carriage:1
- Mate:405: x-carriage:1 ↔ ED3V6:1
- Mate:406: x-carriage-holder:1 ↔ x-carriage:1
- Mate:407: x-carriage-holder:1 ↔ x-carriage:1
- Mate:408: x-carriage-holder:1 ↔ x-carriage:1
- Flush:74: x-carriage:1 ↔ ED3V6:1
- Flush:75: GT2-Pulley-20-Teeth-5mm-Bore:2 ↔ Gt20:2
- Mate:409: x-carriage-2020:1 ↔ X-connectorLeft_MIR:1
- Mate:410: x-carriage-2020:1 ↔ X-connectorLeft:1
- Mate:411 (-27 mm): x-carriage-2020:1 ↔ X-connectorLeft:1
- Mate:415: MGN-12-H-carriage:1 ↔ X-connectorLeft_MIR:1
- Mate:419: Gt20:5 ↔ bracket-GT2-left:1
- Mate:421: x-carriage-2020:1 ↔ holder-GT2-x-carriage-left:1
- Mate:422: x-carriage-2020:1 ↔ holder-GT2-x-carriage-left:1
- Mate:423: Gt20:8 ↔ M5x35mm-crosshead:1
- Mate:424: Gt20:7 ↔ M5x35mm-crosshead:2
- Mate:425: holder-GT2-x-carriage-left:1 ↔ M5x35mm-crosshead:2
- Mate:426: holder-GT2-x-carriage-left:1 ↔ M5x35mm-crosshead:1
- Mate:427: Gt20:8 ↔ M5x35mm-crosshead:1
- Mate:428: M5-nut:7 ↔ M5x35mm-crosshead:1
- Mate:429: holder-GT2-x-carriage-left:1 ↔ M5-nut:7
- Mate:430: M5-nut:8 ↔ M5x35mm-crosshead:2
- Mate:431: holder-GT2-x-carriage-left:1 ↔ M5-nut:8
- Mate:432: x-carriage-2020:1 ↔ holder-GT2-x-carriage-left:1
- Mate:433: Gt20:7 ↔ M5x35mm-crosshead:2
- Flush:76: Gt20:7 ↔ Gt20:6
- Flush:77: Gt20:8 ↔ Gt20:5
- Mate:434: 2020-500mm:1 ↔ 2020-320mm:5
- Mate:435: 2020-320mm:5 ↔ 2020-corner-bracket:30
- Flush:78: 2020-500mm:1 ↔ 2020-320mm:5
- Mate:436: 2020-320mm:5 ↔ 2020-corner-bracket:27
- Flush:79: 2020-350mm:10 ↔ 2020-320mm:5
- Flush:80: 2020-350mm:11 ↔ 2020-320mm:5
- Flush:81: 2020-350mm:11 ↔ 2020-320mm:6
- Mate:437: 2020-320mm:5 ↔ 2020-corner-bracket:26
- Mate:438: 2020-320mm:5 ↔ 2020-corner-bracket:31
- Mate:439: 2020-500mm:2 ↔ 2020-320mm:6
- Mate:440: 2020-320mm:6 ↔ 2020-corner-bracket:24
- Mate:441: 2020-320mm:6 ↔ 2020-corner-bracket:29
- Flush:82: 2020-500mm:3 ↔ 2020-320mm:6
- Mate:442: 2020-320mm:6 ↔ 2020-corner-bracket:22
- Mate:443: 2020-320mm:6 ↔ 2020-corner-bracket:32
- Mate:444: 2020-320mm:5 ↔ 2020-corner-bracket:31
- Mate:445 (45 mm): 2020-320mm:2 ↔ 2020-320mm:6
- Mate:446: 2020-320mm:3 ↔ 2020-corner-bracket:34
- Mate:447: 2020-500mm:4 ↔ 2020-corner-bracket:34
- Mate:448: 2020-320mm:3 ↔ 2020-corner-bracket:34
- Mate:449: 2020-350mm:4 ↔ 2020-corner-bracket:33
- Mate:450: 2020-500mm:4 ↔ 2020-corner-bracket:33
- Mate:452: 2020-350mm:4 ↔ 2020-corner-bracket:1
- Mate:453: 2020-320mm:4 ↔ 2020-corner-bracket:35
- Mate:454: 2020-320mm:4 ↔ 2020-corner-bracket:35
- Mate:455: 2020-500mm:2 ↔ 2020-corner-bracket:35
- Mate:456: 2020-500mm:3 ↔ 2020-corner-bracket:36
- Mate:457: 2020-320mm:4 ↔ 2020-corner-bracket:36
- Mate:458: 2020-320mm:4 ↔ 2020-corner-bracket:36
- Mate:459: 2020-500mm:1 ↔ 2020-corner-bracket:37
- Mate:460: 2020-320mm:3 ↔ 2020-corner-bracket:37
- Mate:461: 2020-320mm:3 ↔ 2020-corner-bracket:37
- Mate:465: e3d titan:1 ↔ mount-extruder:1
- Mate:466: e3d titan:1 ↔ mount-extruder:1
- Mate:467: mount-extruder:1 ↔ nema-17:4
- Mate:468: mount-extruder:1 ↔ nema-17:4
- Mate:469: mount-extruder:1 ↔ nema-17:4
- Mate:470: e3d titan:1 ↔ mount-extruder:1
- Mate:471: 2020-500mm:1 ↔ mount-extruder:1
- Mate:472: 2020-500mm:1 ↔ mount-extruder:1
- Mate:473: 2020-500mm:1 ↔ mount-extruder:1
